# Autodesk Inventor assembly: wheel+hub+motor
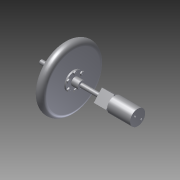
[picture p0: Inventor's stored thumbnail of the model, 180x180]
Saved by Autodesk Inventor 2011 SP1 (Build 150282100, 282)
## iProperties
Created: 2013-01-18
Part Number: wheel+hub+motor
Document SubType Name: Assembly
Designer: wes
Author: wes
## Documents named in this file (7)
- F:\ALL FILES\My Documents\GitHub\2013CAD\2013 robot\CurvedShooter\wheel+hub+axle.iam
- F:\ALL FILES\My Documents\GitHub\2013CAD\2013 robot\CurvedShooter\pneumatic 8'' wheel sketchy quality.ipt
- F:\ALL FILES\My Documents\GitHub\2013CAD\2013 robot\CurvedShooter\Common Chassis Parts\.2'' diameter 2.5 inch bolts for wheel.ipt
- F:\ALL FILES\My Documents\GitHub\2013CAD\2013 robot\CurvedShooter\500-key-hub.ipt
- F:\ALL FILES\My Documents\GitHub\2013CAD\2013 robot\CurvedShooter\key for pneumatic wheel + motor.ipt
- F:\ALL FILES\My Documents\GitHub\2013CAD\2013 robot\CurvedShooter\.5in diameter keyed axle.ipt
- F:\ALL FILES\My Documents\GitHub\2013CAD\2013 robot\CurvedShooter\motor+gbox assembly.iam
## Components (12 placed, 6 different names)
1. pneumatic 8'' wheel sketchy quality:1 — Insert:7, Tangent:1
2. .2'' diameter 2.5 inch bolts for wheel:1 — Insert:1, Tangent:1
3. .2'' diameter 2.5 inch bolts for wheel:2 — Insert:2
4. .2'' diameter 2.5 inch bolts for wheel:3 — Insert:3
5. .2'' diameter 2.5 inch bolts for wheel:4 — Insert:4
6. .2'' diameter 2.5 inch bolts for wheel:5 — Insert:5
7. 500-key-hub:1 — Insert:1, Insert:2, Insert:3, Insert:4, Insert:5, Insert:7, Insert:8, Mate:3, Mate:4, Mate:5, Mate:8, Mate:9
8. key for pneumatic wheel + motor:1 — Mate:3, Mate:4, Mate:5
9. .2'' diameter 2.5 inch bolts for wheel:6 — Insert:8
10. .5in diameter keyed axle:1 — Mate:6, Mate:7, Mate:10, Tangent:2
11. key for pneumatic wheel + motor:2 — Mate:6, Mate:7, Mate:8, Mate:9
12. motor+gbox assembly:1 [sub-assembly] — Mate:10, Tangent:2
## Relationships (17: Mate 8, Insert 7, Tangent 2)
- Insert:1: .2'' diameter 2.5 inch bolts for wheel:1 ↔ 500-key-hub:1
- Insert:2: .2'' diameter 2.5 inch bolts for wheel:2 ↔ 500-key-hub:1
- Insert:3: .2'' diameter 2.5 inch bolts for wheel:3 ↔ 500-key-hub:1
- Insert:4: .2'' diameter 2.5 inch bolts for wheel:4 ↔ 500-key-hub:1
- Insert:5: .2'' diameter 2.5 inch bolts for wheel:5 ↔ 500-key-hub:1
- Insert:7: pneumatic 8'' wheel sketchy quality:1 ↔ 500-key-hub:1
- Insert:8: 500-key-hub:1 ↔ .2'' diameter 2.5 inch bolts for wheel:6
- Tangent:1 (-5.08 mm): pneumatic 8'' wheel sketchy quality:1 ↔ .2'' diameter 2.5 inch bolts for wheel:1
- Mate:3: 500-key-hub:1 ↔ key for pneumatic wheel + motor:1
- Mate:4: 500-key-hub:1 ↔ key for pneumatic wheel + motor:1
- Mate:5 (-44.45 mm): 500-key-hub:1 ↔ key for pneumatic wheel + motor:1
- Mate:6: .5in diameter keyed axle:1 ↔ key for pneumatic wheel + motor:2
- Mate:7: .5in diameter keyed axle:1 ↔ key for pneumatic wheel + motor:2
- Mate:8: 500-key-hub:1 ↔ key for pneumatic wheel + motor:2
- Mate:9: 500-key-hub:1 ↔ key for pneumatic wheel + motor:2
- Mate:10: .5in diameter keyed axle:1 ↔ motor+gbox assembly:1
- Tangent:2: .5in diameter keyed axle:1 ↔ motor+gbox assembly:1
